# Autodesk Inventor assembly: ConveyorFullAssembly
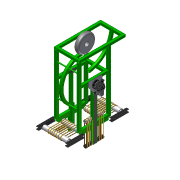
[picture p0: Inventor's stored thumbnail of the model, 180x180]
Saved by Autodesk Inventor 2012 (Build 160160000, 160)
## iProperties
Created: 2012-01-13
Part Number: ConveyorFullAssembly
Document SubType Name: Assembly
Designer: JesseK
Mass: 5863.89 g
Surface Area: 23117.6 cm^2
Volume: 4226.66 cm^3
Density: 1.38736 g/cm^3
Author: JesseK
## Documents named in this file (15)
- Z:\UserData\Documents\Inventor\team1885frc\Robot2012\Conveyor2\ConveyorFullAssembly.iam
- Z:\UserData\Documents\Inventor\team1885frc\Robot2012\Conveyor2\FrameAssembly.iam
- Z:\UserData\Documents\Inventor\team1885frc\Robot2012\Conveyor2\Conveyor_Roller_Cross.ipt
- Z:\UserData\Documents\Inventor\team1885frc\Robot2012\Conveyor2\Belt_Timing_VerticalLongMiddle.ipt
- Z:\UserData\Documents\Inventor\team1885frc\Robot2012\Conveyor2\DriveRoller.iam
- Z:\UserData\Documents\Inventor\team1885frc\Robot2012\Conveyor2\IdleRoller.iam
- Z:\UserData\Documents\Inventor\team1885frc\Robot2012\Conveyor2\Frame_OuterConveyorMount.ipt
- Z:\UserData\Documents\Inventor\team1885frc\Robot2012\Conveyor2\Conveyor_Roller_Outer.ipt
- Z:\UserData\Documents\Inventor\team1885frc\Robot2012\Conveyor2\Belt_Horizontal_Intake.ipt
- Z:\UserData\Documents\Inventor\team1885frc\Robot2012\Conveyor2\ShooterWheelConcept.ipt
- Z:\UserData\Documents\Inventor\team1885frc\Robot2012\Conveyor2\Plate_PictureMountPlate.ipt
- Z:\UserData\Documents\Inventor\team1885frc\KOP Motors\ND Motor Right.iam
- Z:\UserData\Documents\Inventor\team1885frc\Robot2012\Conveyor2\Conveyor_Roller_MainOuter.ipt
- Z:\UserData\Documents\Inventor\team1885frc\KOP Misc\igus bearing mount.iam
- Z:\UserData\Documents\Inventor\team1885frc\Robot2012\Conveyor2\Belt_Vertical_Short.ipt
## Components (38 placed, 14 different names)
1. FrameAssembly:1 [sub-assembly] — Mate:6, Mate:7, Mate:21, Flush:5, Mate:28, Mate:29, Mate:30, Mate:31, Mate:32, Mate:33, Mate:34, Mate:35, Mate:36, Mate:37, Mate:38, Mate:39, Flush:7, Mate:58, Mate:62, Mate:63, Mate:64, Mate:65, Mate:66
2. Conveyor_Roller_Cross:1 — Mate:6, Flush:4, Tangent:6, Tangent:7, Tangent:9, Tangent:10, Tangent:11, Tangent:22, Tangent:23
3. Conveyor_Roller_Cross:2 — Mate:7, Flush:4, Tangent:12, Tangent:13, Tangent:14, Tangent:15, Tangent:16, Tangent:17, Tangent:18, Tangent:19, Tangent:20, Tangent:21
4. DriveRoller:1 [sub-assembly] — Mate:21, Flush:5, Mate:23, Flush:8, Mate:68, Mate:69, Mate:70, Mate:71, Mate:72, Mate:73
5. Belt_Timing_VerticalLongMiddle:1 — Mate:23
6. Frame_OuterConveyorMount:1 — Mate:31, Mate:32, Mate:33, Mate:40
7. Frame_OuterConveyorMount:2 — Mate:28, Mate:29, Mate:30
8. Frame_OuterConveyorMount:3 — Mate:34, Mate:35, Mate:36
9. Frame_OuterConveyorMount:4 — Mate:37, Mate:38, Mate:39, Mate:41
10. Conveyor_Roller_Outer:1 — Mate:40, Mate:42, Mate:43, Mate:45, Mate:46, Mate:47, Mate:48, Mate:49
11. Conveyor_Roller_Outer:2 — Mate:41, Mate:50, Mate:51, Mate:52, Mate:53, Mate:54, Mate:55, Mate:56, Mate:57
12. Belt_Horizontal_Intake:1 — Mate:57, Tangent:12
13. Belt_Horizontal_Intake:2 — Mate:56, Tangent:15
14. Belt_Horizontal_Intake:3 — Mate:55, Tangent:17, Tangent:18, Tangent:21
15. Belt_Horizontal_Intake:4 — Mate:54, Tangent:19
16. Belt_Horizontal_Intake:5 — Mate:53, Tangent:13
17. Belt_Horizontal_Intake:6 — Mate:52, Tangent:14
18. Belt_Horizontal_Intake:7 — Mate:51, Tangent:16
19. Belt_Horizontal_Intake:8 — Mate:50, Tangent:20
20. Belt_Horizontal_Intake:9 — Mate:49, Tangent:6
21. Belt_Horizontal_Intake:10 — Mate:48, Tangent:10
22. Belt_Horizontal_Intake:11 — Mate:47, Tangent:11
23. Belt_Horizontal_Intake:12 — Mate:46, Tangent:23
24. Belt_Horizontal_Intake:13 — Mate:45, Tangent:9
25. Belt_Horizontal_Intake:15 — Mate:43, Tangent:7
26. Belt_Horizontal_Intake:16 — Mate:42, Tangent:22
27. ShooterWheelConcept:1 — Flush:7
28. Plate_PictureMountPlate:1 — Mate:58, Mate:60, Mate:61, Mate:62, Mate:63
29. ND Motor Right:1 [sub-assembly] — Mate:60, Mate:61, Mate:67
30. IdleRoller:2 [sub-assembly] — Mate:64, Flush:8, Tangent:24, Tangent:25, Tangent:26, Tangent:27, Tangent:28, Tangent:29
31. Conveyor_Roller_MainOuter:1 — Mate:65
32. igus bearing mount:1 [sub-assembly] — Mate:66, Mate:67
33. Belt_Vertical_Short:1 — Mate:69, Tangent:24
34. Belt_Vertical_Short:2 — Mate:70, Tangent:25
35. Belt_Vertical_Short:3 — Mate:71, Tangent:29
36. Belt_Vertical_Short:4 — Mate:73, Tangent:27
37. Belt_Vertical_Short:5 — Mate:68, Tangent:26
38. Belt_Vertical_Short:6 — Mate:72, Tangent:28
## Relationships (75: Mate 48, Tangent 23, Flush 4)
- Mate:6: FrameAssembly:1 ↔ Conveyor_Roller_Cross:1
- Mate:7: FrameAssembly:1 ↔ Conveyor_Roller_Cross:2
- Flush:4: Conveyor_Roller_Cross:1 ↔ Conveyor_Roller_Cross:2
- Mate:21: FrameAssembly:1 ↔ DriveRoller:1
- Flush:5 (-76.2 mm): FrameAssembly:1 ↔ DriveRoller:1
- Mate:23: DriveRoller:1 ↔ Belt_Timing_VerticalLongMiddle:1
- Mate:28 (6.35 mm): FrameAssembly:1 ↔ Frame_OuterConveyorMount:2
- Mate:29: FrameAssembly:1 ↔ Frame_OuterConveyorMount:2
- Mate:30: FrameAssembly:1 ↔ Frame_OuterConveyorMount:2
- Mate:31 (6.35 mm): FrameAssembly:1 ↔ Frame_OuterConveyorMount:1
- Mate:32: FrameAssembly:1 ↔ Frame_OuterConveyorMount:1
- Mate:33: FrameAssembly:1 ↔ Frame_OuterConveyorMount:1
- Mate:34 (6.35 mm): FrameAssembly:1 ↔ Frame_OuterConveyorMount:3
- Mate:35: FrameAssembly:1 ↔ Frame_OuterConveyorMount:3
- Mate:36: FrameAssembly:1 ↔ Frame_OuterConveyorMount:3
- Mate:37 (6.35 mm): FrameAssembly:1 ↔ Frame_OuterConveyorMount:4
- Mate:38: FrameAssembly:1 ↔ Frame_OuterConveyorMount:4
- Mate:39: FrameAssembly:1 ↔ Frame_OuterConveyorMount:4
- Mate:40: Frame_OuterConveyorMount:1 ↔ Conveyor_Roller_Outer:1
- Mate:41: Frame_OuterConveyorMount:4 ↔ Conveyor_Roller_Outer:2
- Mate:42: Conveyor_Roller_Outer:1 ↔ Belt_Horizontal_Intake:16
- Mate:43: Conveyor_Roller_Outer:1 ↔ Belt_Horizontal_Intake:15
- Mate:45: Conveyor_Roller_Outer:1 ↔ Belt_Horizontal_Intake:13
- Mate:46: Conveyor_Roller_Outer:1 ↔ Belt_Horizontal_Intake:12
- Mate:47: Conveyor_Roller_Outer:1 ↔ Belt_Horizontal_Intake:11
- Mate:48: Conveyor_Roller_Outer:1 ↔ Belt_Horizontal_Intake:10
- Mate:49: Conveyor_Roller_Outer:1 ↔ Belt_Horizontal_Intake:9
- Mate:50: Conveyor_Roller_Outer:2 ↔ Belt_Horizontal_Intake:8
- Mate:51: Conveyor_Roller_Outer:2 ↔ Belt_Horizontal_Intake:7
- Mate:52: Conveyor_Roller_Outer:2 ↔ Belt_Horizontal_Intake:6
- Mate:53: Conveyor_Roller_Outer:2 ↔ Belt_Horizontal_Intake:5
- Mate:54: Conveyor_Roller_Outer:2 ↔ Belt_Horizontal_Intake:4
- Mate:55: Conveyor_Roller_Outer:2 ↔ Belt_Horizontal_Intake:3
- Mate:56: Conveyor_Roller_Outer:2 ↔ Belt_Horizontal_Intake:2
- Mate:57: Conveyor_Roller_Outer:2 ↔ Belt_Horizontal_Intake:1
- Tangent:6: Conveyor_Roller_Cross:1 ↔ Belt_Horizontal_Intake:9
- Tangent:7: Conveyor_Roller_Cross:1 ↔ Belt_Horizontal_Intake:15
- Tangent:9: Conveyor_Roller_Cross:1 ↔ Belt_Horizontal_Intake:13
- Tangent:10: Conveyor_Roller_Cross:1 ↔ Belt_Horizontal_Intake:10
- Tangent:11: Conveyor_Roller_Cross:1 ↔ Belt_Horizontal_Intake:11
- Tangent:12: Conveyor_Roller_Cross:2 ↔ Belt_Horizontal_Intake:1
- Tangent:13: Conveyor_Roller_Cross:2 ↔ Belt_Horizontal_Intake:5
- Tangent:14: Conveyor_Roller_Cross:2 ↔ Belt_Horizontal_Intake:6
- Tangent:15: Conveyor_Roller_Cross:2 ↔ Belt_Horizontal_Intake:2
- Tangent:16: Conveyor_Roller_Cross:2 ↔ Belt_Horizontal_Intake:7
- Tangent:17: Conveyor_Roller_Cross:2 ↔ Belt_Horizontal_Intake:3
- Tangent:18: Conveyor_Roller_Cross:2 ↔ Belt_Horizontal_Intake:3
- Tangent:19: Conveyor_Roller_Cross:2 ↔ Belt_Horizontal_Intake:4
- Tangent:20: Conveyor_Roller_Cross:2 ↔ Belt_Horizontal_Intake:8
- Tangent:21: Conveyor_Roller_Cross:2 ↔ Belt_Horizontal_Intake:3
- Tangent:22: Conveyor_Roller_Cross:1 ↔ Belt_Horizontal_Intake:16
- Tangent:23: Conveyor_Roller_Cross:1 ↔ Belt_Horizontal_Intake:12
- Flush:7 (114.3 mm): FrameAssembly:1 ↔ ShooterWheelConcept:1
- Mate:58: FrameAssembly:1 ↔ Plate_PictureMountPlate:1
- Mate:60 (2.54 mm): Plate_PictureMountPlate:1 ↔ ND Motor Right:1
- Mate:61: Plate_PictureMountPlate:1 ↔ ND Motor Right:1
- Mate:62 (-50.8 mm): FrameAssembly:1 ↔ Plate_PictureMountPlate:1
- Mate:63: FrameAssembly:1 ↔ Plate_PictureMountPlate:1
- Mate:64: FrameAssembly:1 ↔ IdleRoller:2
- Flush:8: DriveRoller:1 ↔ IdleRoller:2
- Mate:65: FrameAssembly:1 ↔ Conveyor_Roller_MainOuter:1
- Mate:66: FrameAssembly:1 ↔ igus bearing mount:1
- Mate:67: ND Motor Right:1 ↔ igus bearing mount:1
- Mate:68: DriveRoller:1 ↔ Belt_Vertical_Short:5
- Mate:69: DriveRoller:1 ↔ Belt_Vertical_Short:1
- Mate:70: DriveRoller:1 ↔ Belt_Vertical_Short:2
- Mate:71: DriveRoller:1 ↔ Belt_Vertical_Short:3
- Mate:72: DriveRoller:1 ↔ Belt_Vertical_Short:6
- Mate:73: DriveRoller:1 ↔ Belt_Vertical_Short:4
- Tangent:24: IdleRoller:2 ↔ Belt_Vertical_Short:1
- Tangent:25: IdleRoller:2 ↔ Belt_Vertical_Short:2
- Tangent:26: IdleRoller:2 ↔ Belt_Vertical_Short:5
- Tangent:27: IdleRoller:2 ↔ Belt_Vertical_Short:4
- Tangent:28: IdleRoller:2 ↔ Belt_Vertical_Short:6
- Tangent:29: IdleRoller:2 ↔ Belt_Vertical_Short:3
